# Autodesk Inventor assembly: Hepheaestes38v2 1
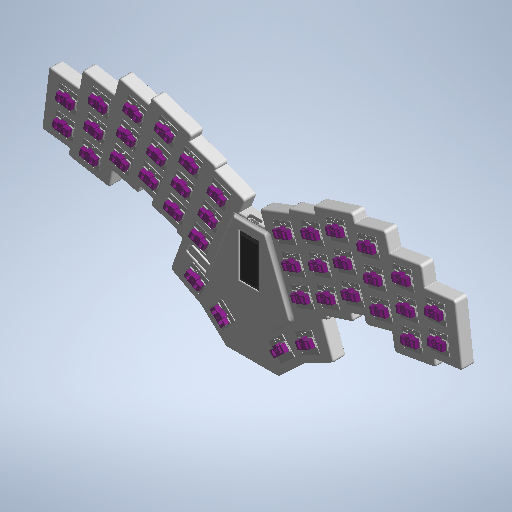
[picture p0: Inventor's stored thumbnail of the model, 512x512]
Saved by Autodesk Inventor 2025 (Build 290162000, 162)
## iProperties
Company: Kicad
Created: 2025-11-22
Part Number: Hepheaestes38v2 1
Description: KiCad electronic assembly
Document SubType Name: Assembly
Designer: User
Authority: Unknown
Mass: 156.593 g
Surface Area: 2055.32 cm^2
Volume: 126.592 cm^3
Density: 1.23699 g/cm^3
Sending System: KiCad to STEP converter
Preprocessor: Open CASCADE STEP processor 7.9
Title: Hepheaestes38v2.step
Author: Pcbnew
## Documents named in this file (18)
- C:\Users\User\Hephaestes38-zmk\PCB, Case\Case V2\Hepheaestes38v2 CAD\Hepheaestes38v2.iam
- C:\Users\User\Hephaestes38-zmk\PCB, Case\Case V2\Hepheaestes38v2 CAD\Hepheaestes38v2_copper.ipt
- C:\Users\User\Hephaestes38-zmk\PCB, Case\Case V2\Hepheaestes38v2 CAD\Hepheaestes38v2_pad.ipt
- C:\Users\User\Hephaestes38-zmk\PCB, Case\Case V2\Hepheaestes38v2 CAD\Hepheaestes38v2_via.ipt
- C:\Users\User\Hephaestes38-zmk\PCB, Case\Case V2\Hepheaestes38v2 CAD\Hepheaestes38v2_silkscreen.ipt
- C:\Users\User\Hephaestes38-zmk\PCB, Case\Case V2\Hepheaestes38v2 CAD\Hepheaestes38v2_PCB.ipt
- C:\Users\User\Hephaestes38-zmk\PCB, Case\Case V2\Hepheaestes38v2 CAD\Nice Nano V2.iam
- C:\Users\User\Hephaestes38-zmk\PCB, Case\Case V2\Hepheaestes38v2 CAD\nice!view\nice!view.ipt
- C:\Users\User\Documents\Inventor\Content Center Files\R2025\en-US\BS EN ISO 7045 Z\EN ISO 7045 - M2 x 5 - 4.8 - Z(1).ipt
- C:\Users\User\Hephaestes38-zmk\PCB, Case\Case V2\Hepheaestes38v2 CAD\PCM12SMTR_PART1.ipt
- C:\Users\User\Hephaestes38-zmk\PCB, Case\Case V2\Hepheaestes38v2 CAD\PTS526 Reset button.ipt
- C:\Users\User\Hephaestes38-zmk\PCB, Case\Case V2\Hepheaestes38v2 CAD\Kailh Choc Hotswap Socket.ipt
- C:\Users\User\Hephaestes38-zmk\PCB, Case\Case V2\Hephaestus38v2 Case Top.ipt
- C:\Users\User\Hephaestes38-zmk\PCB, Case\Case V2\Hephaestus38v2 Case Bottom.ipt
- C:\Users\User\Hephaestes38-zmk\PCB, Case\Case V2\Hephaestus38v2 Switchplate.ipt
- C:\Users\User\Hephaestes38-zmk\PCB, Case\Case V2\Hepheaestes38v2 CAD\S2B-PH-K-S.ipt
- C:\Users\User\Hephaestes38-zmk\PCB, Case\Case V2\Hepheaestes38v2 CAD\Kailh LP Choc Purpz.ipt
- C:\Users\User\Hephaestes38-zmk\PCB, Case\Case V2\Hephaestus38v2 Case Screen Cover.ipt
## Components (100 placed, 17 different names)
1. Nice Nano V2:1 [sub-assembly] — Mate:1, Mate:2, Mate:3
2. nice!view:1 — Mate:4, Mate:5, Mate:6
3. PCM12SMTR_PART1:1 — Mate:60, Mate:61, Mate:62
4. PTS526 Reset button:1 — Mate:63, Flush:1, Flush:2
5. S2B-PH-K-S:1 — Mate:183, Tangent:1
6. Hephaestus38v2 Case Top:1 — Mate:55, Mate:58, Mate:59, Mate:184, Mate:187, Mate:188
7. Hephaestus38v2 Case Bottom:1 — Flush:3, Insert:35, Insert:36, Insert:37, Insert:38, Insert:39, Insert:40, Insert:41, Insert:42, Insert:43, Insert:44
8. Hephaestus38v2 Switchplate:1 — Mate:182, Flush:4, Flush:5
9. Hephaestus38v2 Case Screen Cover:1 — Mate:184, Mate:187, Mate:188
10. 1
11. 2 — Mate:2, Mate:3, Mate:5, Mate:6, Flush:1, Flush:2, Mate:67, Mate:70, Mate:73, Mate:76, Mate:79, Mate:82, Mate:85, Mate:88, Mate:91, Mate:94, Mate:97, Mate:100, Mate:103, Mate:106, Mate:109, Mate:112, Mate:115, Mate:118, Mate:121, Mate:124, Mate:127, Mate:130, Mate:133, Mate:136, Mate:139, Mate:142, Mate:145, Mate:148, Mate:151, Mate:154, Mate:157, Mate:160, Mate:163, Mate:166, Mate:169, Mate:172, Mate:175, Mate:178, Tangent:1
12. 3
13. 4
14. 5 — Mate:1, Mate:4, Mate:7, Mate:8, Mate:9, Mate:10, Mate:11, Mate:12, Insert:1, Insert:2, Insert:3, Insert:4, Insert:5, Insert:6, Insert:7, Insert:8, Insert:9, Insert:10, Insert:11, Insert:12, Insert:13, Insert:14, Mate:13, Mate:14, Mate:15, Mate:16, Mate:17, Mate:18, Mate:19, Mate:20, Mate:21, Mate:22, Mate:23, Mate:24, Mate:25, Mate:26, Insert:15, Insert:16, Insert:17, Insert:18, Insert:19, Mate:28, Insert:20, Insert:22, Insert:23, Insert:21, Mate:29, Mate:30, Mate:31, Mate:32, Mate:33, Mate:34, Mate:35, Mate:36, Mate:37, Mate:38, Mate:39, Mate:40, Mate:41, Mate:42, Insert:24, Insert:25, Insert:26, Insert:27, Insert:28, Insert:29, Insert:30, Insert:31, Insert:32, Insert:33, Insert:34, Mate:43, Mate:44, Mate:45, Mate:46, Mate:47, Mate:48, Mate:49, Mate:50, Mate:51, Mate:52, Mate:53, Mate:55, Mate:58, Mate:59, Mate:60, Mate:61, Mate:62, Mate:63, Mate:65, Mate:66, Mate:68, Mate:69, Mate:71, Mate:72, Mate:74, Mate:75, Mate:77, Mate:78, Mate:80, Mate:81, Mate:83, Mate:84, Mate:86, Mate:87, Mate:89, Mate:90, Mate:92, Mate:93, Mate:95, Mate:96, Mate:98, Mate:99, Mate:101, Mate:102, Mate:104, Mate:105, Mate:107, Mate:108, Mate:110, Mate:111, Mate:113, Mate:114, Mate:116, Mate:117, Mate:119, Mate:120, Mate:122, Mate:123, Mate:125, Mate:126, Mate:128, Mate:129, Mate:131, Mate:132, Mate:134, Mate:135, Mate:137, Mate:138, Mate:140, Mate:141, Mate:143, Mate:144, Mate:146, Mate:147, Mate:149, Mate:150, Mate:152, Mate:153, Mate:155, Mate:156, Mate:158, Mate:159, Mate:161, Mate:162, Mate:164, Mate:165, Mate:167, Mate:168, Mate:170, Mate:171, Mate:173, Mate:174, Mate:176, Mate:177, Insert:45, Mate:183, Flush:4, Flush:5
15. Kailh Choc Hotswap Socket:1 — Mate:65, Mate:66, Mate:67
16. Kailh Choc Hotswap Socket:2 — Mate:68, Mate:69, Mate:70
17. Kailh Choc Hotswap Socket:3 — Mate:74, Mate:75, Mate:76
18. Kailh Choc Hotswap Socket:4 — Mate:77, Mate:78, Mate:79
19. Kailh Choc Hotswap Socket:5 — Mate:71, Mate:72, Mate:73
20. Kailh Choc Hotswap Socket:6 — Mate:83, Mate:84, Mate:85
21. Kailh Choc Hotswap Socket:7 — Mate:89, Mate:90, Mate:91
22. Kailh Choc Hotswap Socket:8 — Mate:80, Mate:81, Mate:82
23. Kailh Choc Hotswap Socket:9 — Mate:86, Mate:87, Mate:88
24. Kailh Choc Hotswap Socket:10 — Mate:92, Mate:93, Mate:94
25. Kailh Choc Hotswap Socket:11 — Mate:95, Mate:96, Mate:97
26. Kailh Choc Hotswap Socket:12 — Mate:98, Mate:99, Mate:100
27. Kailh Choc Hotswap Socket:13 — Mate:101, Mate:102, Mate:103
28. Kailh Choc Hotswap Socket:14 — Mate:104, Mate:105, Mate:106
29. Kailh Choc Hotswap Socket:15 — Mate:107, Mate:108, Mate:109
30. Kailh Choc Hotswap Socket:16 — Mate:110, Mate:111, Mate:112
31. Kailh Choc Hotswap Socket:17 — Mate:113, Mate:114, Mate:115, Flush:3
32. Kailh Choc Hotswap Socket:18 — Mate:116, Mate:117, Mate:118
33. Kailh Choc Hotswap Socket:19 — Mate:119, Mate:120, Mate:121
34. Kailh Choc Hotswap Socket:20 — Mate:122, Mate:123, Mate:124
35. Kailh Choc Hotswap Socket:21 — Mate:125, Mate:126, Mate:127
36. Kailh Choc Hotswap Socket:22 — Mate:128, Mate:129, Mate:130
37. Kailh Choc Hotswap Socket:23 — Mate:131, Mate:132, Mate:133
38. Kailh Choc Hotswap Socket:24 — Mate:134, Mate:135, Mate:136
39. Kailh Choc Hotswap Socket:25 — Mate:137, Mate:138, Mate:139
40. Kailh Choc Hotswap Socket:26 — Mate:140, Mate:141, Mate:142
41. Kailh Choc Hotswap Socket:27 — Mate:143, Mate:144, Mate:145
42. Kailh Choc Hotswap Socket:28 — Mate:146, Mate:147, Mate:148
43. Kailh Choc Hotswap Socket:29 — Mate:155, Mate:156, Mate:157
44. Kailh Choc Hotswap Socket:30 — Mate:152, Mate:153, Mate:154
45. Kailh Choc Hotswap Socket:31 — Mate:149, Mate:150, Mate:151
46. Kailh Choc Hotswap Socket:32 — Mate:161, Mate:162, Mate:163
47. Kailh Choc Hotswap Socket:33 — Mate:164, Mate:165, Mate:166
48. Kailh Choc Hotswap Socket:34 — Mate:167, Mate:168, Mate:169
49. Kailh Choc Hotswap Socket:35 — Mate:170, Mate:171, Mate:172
50. Kailh Choc Hotswap Socket:36 — Mate:158, Mate:159, Mate:160
51. Kailh Choc Hotswap Socket:37 — Mate:173, Mate:174, Mate:175
52. Kailh Choc Hotswap Socket:38 — Mate:176, Mate:177, Mate:178
53. Kailh LP Choc Purpz:1 — Mate:7, Mate:8, Mate:9, Mate:34
54. Kailh LP Choc Purpz:2 — Insert:1, Mate:13
55. Kailh LP Choc Purpz:3 — Mate:10, Mate:11, Mate:12
56. Kailh LP Choc Purpz:4 — Insert:2, Mate:14, Mate:35
57. Kailh LP Choc Purpz:5 — Insert:3, Mate:15, Mate:40
58. Kailh LP Choc Purpz:6 — Insert:4, Mate:16
59. Kailh LP Choc Purpz:7 — Insert:5, Mate:17
60. Kailh LP Choc Purpz:8 — Insert:6, Mate:18
61. Kailh LP Choc Purpz:9 — Insert:7, Mate:19
62. Kailh LP Choc Purpz:10 — Insert:8, Mate:20
63. Kailh LP Choc Purpz:11 — Insert:9, Mate:21
64. Kailh LP Choc Purpz:12 — Insert:10, Mate:22
65. Kailh LP Choc Purpz:13 — Insert:14, Mate:23
66. Kailh LP Choc Purpz:14 — Insert:13, Mate:24
67. Kailh LP Choc Purpz:15 — Insert:12, Mate:25
68. Kailh LP Choc Purpz:16 — Insert:11, Mate:26
69. Kailh LP Choc Purpz:17 — Insert:16, Mate:31
70. Kailh LP Choc Purpz:18 — Insert:23, Mate:30
71. Kailh LP Choc Purpz:19 — Insert:15, Mate:29, Mate:182
72. Kailh LP Choc Purpz:20 — Insert:17, Mate:33
73. Kailh LP Choc Purpz:21 — Insert:18, Mate:36
74. Kailh LP Choc Purpz:22 — Insert:19, Mate:39
75. Kailh LP Choc Purpz:23 — Insert:21, Mate:37
76. Kailh LP Choc Purpz:24 — Insert:22, Mate:32
77. Kailh LP Choc Purpz:25 — Insert:20, Mate:38
78. Kailh LP Choc Purpz:26 — Mate:28, Mate:42
79. Kailh LP Choc Purpz:27 — Mate:41, Insert:45
80. Kailh LP Choc Purpz:28 — Insert:30, Mate:44
81. Kailh LP Choc Purpz:29 — Insert:27, Mate:52
82. Kailh LP Choc Purpz:30 — Insert:24, Mate:49
83. Kailh LP Choc Purpz:31 — Insert:32, Mate:46
84. Kailh LP Choc Purpz:32 — Insert:33, Mate:47
85. Kailh LP Choc Purpz:33 — Insert:34, Mate:48
86. Kailh LP Choc Purpz:34 — Insert:28, Mate:53
87. Kailh LP Choc Purpz:35 — Insert:26, Mate:51
88. Kailh LP Choc Purpz:36 — Insert:25, Mate:50
89. Kailh LP Choc Purpz:37 — Insert:29, Mate:43
90. Kailh LP Choc Purpz:38 — Insert:31, Mate:45
91. BS EN ISO 7045 Z - Metric M2 x 5 - 4.8 - Z:1 — Insert:35
92. BS EN ISO 7045 Z - Metric M2 x 5 - 4.8 - Z:2 — Insert:36
93. BS EN ISO 7045 Z - Metric M2 x 5 - 4.8 - Z:3 — Insert:37
94. BS EN ISO 7045 Z - Metric M2 x 5 - 4.8 - Z:4 — Insert:38
95. BS EN ISO 7045 Z - Metric M2 x 5 - 4.8 - Z:5 — Insert:39
96. BS EN ISO 7045 Z - Metric M2 x 5 - 4.8 - Z:6 — Insert:40
97. BS EN ISO 7045 Z - Metric M2 x 5 - 4.8 - Z:7 — Insert:41
98. BS EN ISO 7045 Z - Metric M2 x 5 - 4.8 - Z:8 — Insert:42
99. BS EN ISO 7045 Z - Metric M2 x 5 - 4.8 - Z:9 — Insert:43
100. BS EN ISO 7045 Z - Metric M2 x 5 - 4.8 - Z:10 — Insert:44
## Relationships (229: Mate 178, Insert 45, Flush 5, Tangent 1)
- Mate:1 (2.54 mm): Nice Nano V2:1 ↔ 5
- Mate:2: Nice Nano V2:1 ↔ 2
- Mate:3: Nice Nano V2:1 ↔ 2
- Mate:4 (5.08 mm): nice!view:1 ↔ 5
- Mate:5: nice!view:1 ↔ 2
- Mate:6: nice!view:1 ↔ 2
- Mate:7: 5 ↔ Kailh LP Choc Purpz:1
- Mate:8: 5 ↔ Kailh LP Choc Purpz:1
- Mate:9: 5 ↔ Kailh LP Choc Purpz:1
- Mate:10: 5 ↔ Kailh LP Choc Purpz:3
- Mate:11: 5 ↔ Kailh LP Choc Purpz:3
- Mate:12: 5 ↔ Kailh LP Choc Purpz:3
- Insert:1: 5 ↔ Kailh LP Choc Purpz:2
- Insert:2: 5 ↔ Kailh LP Choc Purpz:4
- Insert:3: 5 ↔ Kailh LP Choc Purpz:5
- Insert:4: 5 ↔ Kailh LP Choc Purpz:6
- Insert:5: 5 ↔ Kailh LP Choc Purpz:7
- Insert:6: 5 ↔ Kailh LP Choc Purpz:8
- Insert:7: 5 ↔ Kailh LP Choc Purpz:9
- Insert:8: 5 ↔ Kailh LP Choc Purpz:10
- Insert:9: 5 ↔ Kailh LP Choc Purpz:11
- Insert:10: 5 ↔ Kailh LP Choc Purpz:12
- Insert:11: 5 ↔ Kailh LP Choc Purpz:16
- Insert:12: 5 ↔ Kailh LP Choc Purpz:15
- Insert:13: 5 ↔ Kailh LP Choc Purpz:14
- Insert:14: 5 ↔ Kailh LP Choc Purpz:13
- Mate:13: 5 ↔ Kailh LP Choc Purpz:2
- Mate:14: 5 ↔ Kailh LP Choc Purpz:4
- Mate:15: 5 ↔ Kailh LP Choc Purpz:5
- Mate:16: 5 ↔ Kailh LP Choc Purpz:6
- Mate:17: 5 ↔ Kailh LP Choc Purpz:7
- Mate:18: 5 ↔ Kailh LP Choc Purpz:8
- Mate:19: 5 ↔ Kailh LP Choc Purpz:9
- Mate:20: 5 ↔ Kailh LP Choc Purpz:10
- Mate:21: 5 ↔ Kailh LP Choc Purpz:11
- Mate:22: 5 ↔ Kailh LP Choc Purpz:12
- Mate:23: 5 ↔ Kailh LP Choc Purpz:13
- Mate:24: 5 ↔ Kailh LP Choc Purpz:14
- Mate:25: 5 ↔ Kailh LP Choc Purpz:15
- Mate:26: 5 ↔ Kailh LP Choc Purpz:16
- Insert:15: 5 ↔ Kailh LP Choc Purpz:19
- Insert:16: 5 ↔ Kailh LP Choc Purpz:17
- Insert:17: 5 ↔ Kailh LP Choc Purpz:20
- Insert:18: 5 ↔ Kailh LP Choc Purpz:21
- Insert:19: 5 ↔ Kailh LP Choc Purpz:22
- Mate:28: 5 ↔ Kailh LP Choc Purpz:26
- Insert:20: 5 ↔ Kailh LP Choc Purpz:25
- Insert:21: 5 ↔ Kailh LP Choc Purpz:23
- Insert:22: 5 ↔ Kailh LP Choc Purpz:24
- Insert:23: 5 ↔ Kailh LP Choc Purpz:18
- Mate:29: 5 ↔ Kailh LP Choc Purpz:19
- Mate:30: 5 ↔ Kailh LP Choc Purpz:18
- Mate:31: 5 ↔ Kailh LP Choc Purpz:17
- Mate:32: 5 ↔ Kailh LP Choc Purpz:24
- Mate:33: 5 ↔ Kailh LP Choc Purpz:20
- Mate:34: 5 ↔ Kailh LP Choc Purpz:1
- Mate:35: 5 ↔ Kailh LP Choc Purpz:4
- Mate:36: 5 ↔ Kailh LP Choc Purpz:21
- Mate:37: 5 ↔ Kailh LP Choc Purpz:23
- Mate:38: 5 ↔ Kailh LP Choc Purpz:25
- Mate:39: 5 ↔ Kailh LP Choc Purpz:22
- Mate:40: 5 ↔ Kailh LP Choc Purpz:5
- Mate:41: 5 ↔ Kailh LP Choc Purpz:27
- Mate:42: 5 ↔ Kailh LP Choc Purpz:26
- Insert:24: 5 ↔ Kailh LP Choc Purpz:30
- Insert:25: 5 ↔ Kailh LP Choc Purpz:36
- Insert:26: 5 ↔ Kailh LP Choc Purpz:35
- Insert:27: 5 ↔ Kailh LP Choc Purpz:29
- Insert:28: 5 ↔ Kailh LP Choc Purpz:34
- Insert:29: 5 ↔ Kailh LP Choc Purpz:37
- Insert:30: 5 ↔ Kailh LP Choc Purpz:28
- Insert:31: 5 ↔ Kailh LP Choc Purpz:38
- Insert:32: 5 ↔ Kailh LP Choc Purpz:31
- Insert:33: 5 ↔ Kailh LP Choc Purpz:32
- Insert:34: 5 ↔ Kailh LP Choc Purpz:33
- Mate:43: 5 ↔ Kailh LP Choc Purpz:37
- Mate:44: 5 ↔ Kailh LP Choc Purpz:28
- Mate:45: 5 ↔ Kailh LP Choc Purpz:38
- Mate:46: 5 ↔ Kailh LP Choc Purpz:31
- Mate:47: 5 ↔ Kailh LP Choc Purpz:32
- Mate:48: 5 ↔ Kailh LP Choc Purpz:33
- Mate:49: 5 ↔ Kailh LP Choc Purpz:30
- Mate:50: 5 ↔ Kailh LP Choc Purpz:36
- Mate:51: 5 ↔ Kailh LP Choc Purpz:35
- Mate:52: 5 ↔ Kailh LP Choc Purpz:29
- Mate:53: 5 ↔ Kailh LP Choc Purpz:34
- Mate:55: Hephaestus38v2 Case Top:1 ↔ 5
- Mate:58: Hephaestus38v2 Case Top:1 ↔ 5
- Mate:59: Hephaestus38v2 Case Top:1 ↔ 5
- Mate:60: PCM12SMTR_PART1:1 ↔ 5
- Mate:61: PCM12SMTR_PART1:1 ↔ 5
- Mate:62: PCM12SMTR_PART1:1 ↔ 5
- Mate:63: PTS526 Reset button:1 ↔ 5
- Flush:1 (0.5 mm): PTS526 Reset button:1 ↔ 2
- Flush:2 (1 mm): PTS526 Reset button:1 ↔ 2
- Mate:65: 5 ↔ Kailh Choc Hotswap Socket:1
- Mate:66: 5 ↔ Kailh Choc Hotswap Socket:1
- Mate:67: 2 ↔ Kailh Choc Hotswap Socket:1
- Mate:68: 5 ↔ Kailh Choc Hotswap Socket:2
- Mate:69: 5 ↔ Kailh Choc Hotswap Socket:2
- Mate:70: 2 ↔ Kailh Choc Hotswap Socket:2
- Mate:71: 5 ↔ Kailh Choc Hotswap Socket:5
- Mate:72: 5 ↔ Kailh Choc Hotswap Socket:5
- Mate:73: 2 ↔ Kailh Choc Hotswap Socket:5
- Mate:74: 5 ↔ Kailh Choc Hotswap Socket:3
- Mate:75: 5 ↔ Kailh Choc Hotswap Socket:3
- Mate:76: 2 ↔ Kailh Choc Hotswap Socket:3
- Mate:77: 5 ↔ Kailh Choc Hotswap Socket:4
- Mate:78: 5 ↔ Kailh Choc Hotswap Socket:4
- Mate:79: 2 ↔ Kailh Choc Hotswap Socket:4
- Mate:80: 5 ↔ Kailh Choc Hotswap Socket:8
- Mate:81: 5 ↔ Kailh Choc Hotswap Socket:8
- Mate:82: 2 ↔ Kailh Choc Hotswap Socket:8
- Mate:83: 5 ↔ Kailh Choc Hotswap Socket:6
- Mate:84: 5 ↔ Kailh Choc Hotswap Socket:6
- Mate:85: 2 ↔ Kailh Choc Hotswap Socket:6
- Mate:86: 5 ↔ Kailh Choc Hotswap Socket:9
- Mate:87: 5 ↔ Kailh Choc Hotswap Socket:9
- Mate:88: 2 ↔ Kailh Choc Hotswap Socket:9
- Mate:89: 5 ↔ Kailh Choc Hotswap Socket:7
- Mate:90: 5 ↔ Kailh Choc Hotswap Socket:7
- Mate:91: 2 ↔ Kailh Choc Hotswap Socket:7
- Mate:92: 5 ↔ Kailh Choc Hotswap Socket:10
- Mate:93: 5 ↔ Kailh Choc Hotswap Socket:10
- Mate:94: 2 ↔ Kailh Choc Hotswap Socket:10
- Mate:95: 5 ↔ Kailh Choc Hotswap Socket:11
- Mate:96: 5 ↔ Kailh Choc Hotswap Socket:11
- Mate:97: 2 ↔ Kailh Choc Hotswap Socket:11
- Mate:98: 5 ↔ Kailh Choc Hotswap Socket:12
- Mate:99: 5 ↔ Kailh Choc Hotswap Socket:12
- Mate:100: 2 ↔ Kailh Choc Hotswap Socket:12
- Mate:101: 5 ↔ Kailh Choc Hotswap Socket:13
- Mate:102: 5 ↔ Kailh Choc Hotswap Socket:13
- Mate:103: 2 ↔ Kailh Choc Hotswap Socket:13
- Mate:104: 5 ↔ Kailh Choc Hotswap Socket:14
- Mate:105: 5 ↔ Kailh Choc Hotswap Socket:14
- Mate:106: 2 ↔ Kailh Choc Hotswap Socket:14
- Mate:107: 5 ↔ Kailh Choc Hotswap Socket:15
- Mate:108: 5 ↔ Kailh Choc Hotswap Socket:15
- Mate:109: 2 ↔ Kailh Choc Hotswap Socket:15
- Mate:110: 5 ↔ Kailh Choc Hotswap Socket:16
- Mate:111: 5 ↔ Kailh Choc Hotswap Socket:16
- Mate:112: 2 ↔ Kailh Choc Hotswap Socket:16
- Mate:113: 5 ↔ Kailh Choc Hotswap Socket:17
- Mate:114: 5 ↔ Kailh Choc Hotswap Socket:17
- Mate:115: 2 ↔ Kailh Choc Hotswap Socket:17
- Mate:116: 5 ↔ Kailh Choc Hotswap Socket:18
- Mate:117: 5 ↔ Kailh Choc Hotswap Socket:18
- Mate:118: 2 ↔ Kailh Choc Hotswap Socket:18
- Mate:119: 5 ↔ Kailh Choc Hotswap Socket:19
- Mate:120: 5 ↔ Kailh Choc Hotswap Socket:19
- Mate:121: 2 ↔ Kailh Choc Hotswap Socket:19
- Mate:122: 5 ↔ Kailh Choc Hotswap Socket:20
- Mate:123: 5 ↔ Kailh Choc Hotswap Socket:20
- Mate:124: 2 ↔ Kailh Choc Hotswap Socket:20
- Mate:125: 5 ↔ Kailh Choc Hotswap Socket:21
- Mate:126: 5 ↔ Kailh Choc Hotswap Socket:21
- Mate:127: 2 ↔ Kailh Choc Hotswap Socket:21
- Mate:128: 5 ↔ Kailh Choc Hotswap Socket:22
- Mate:129: 5 ↔ Kailh Choc Hotswap Socket:22
- Mate:130: 2 ↔ Kailh Choc Hotswap Socket:22
- Mate:131: 5 ↔ Kailh Choc Hotswap Socket:23
- Mate:132: 5 ↔ Kailh Choc Hotswap Socket:23
- Mate:133: 2 ↔ Kailh Choc Hotswap Socket:23
- Mate:134: 5 ↔ Kailh Choc Hotswap Socket:24
- Mate:135: 5 ↔ Kailh Choc Hotswap Socket:24
- Mate:136: 2 ↔ Kailh Choc Hotswap Socket:24
- Mate:137: 5 ↔ Kailh Choc Hotswap Socket:25
- Mate:138: 5 ↔ Kailh Choc Hotswap Socket:25
- Mate:139: 2 ↔ Kailh Choc Hotswap Socket:25
- Mate:140: 5 ↔ Kailh Choc Hotswap Socket:26
- Mate:141: 5 ↔ Kailh Choc Hotswap Socket:26
- Mate:142: 2 ↔ Kailh Choc Hotswap Socket:26
- Mate:143: 5 ↔ Kailh Choc Hotswap Socket:27
- Mate:144: 5 ↔ Kailh Choc Hotswap Socket:27
- Mate:145: 2 ↔ Kailh Choc Hotswap Socket:27
- Mate:146: 5 ↔ Kailh Choc Hotswap Socket:28
- Mate:147: 5 ↔ Kailh Choc Hotswap Socket:28
- Mate:148: 2 ↔ Kailh Choc Hotswap Socket:28
- Mate:149: 5 ↔ Kailh Choc Hotswap Socket:31
- Mate:150: 5 ↔ Kailh Choc Hotswap Socket:31
- Mate:151: 2 ↔ Kailh Choc Hotswap Socket:31
- Mate:152: 5 ↔ Kailh Choc Hotswap Socket:30
- Mate:153: 5 ↔ Kailh Choc Hotswap Socket:30
- Mate:154: 2 ↔ Kailh Choc Hotswap Socket:30
- Mate:155: 5 ↔ Kailh Choc Hotswap Socket:29
- Mate:156: 5 ↔ Kailh Choc Hotswap Socket:29
- Mate:157: 2 ↔ Kailh Choc Hotswap Socket:29
- Mate:158: 5 ↔ Kailh Choc Hotswap Socket:36
- Mate:159: 5 ↔ Kailh Choc Hotswap Socket:36
- Mate:160: 2 ↔ Kailh Choc Hotswap Socket:36
- Mate:161: 5 ↔ Kailh Choc Hotswap Socket:32
- Mate:162: 5 ↔ Kailh Choc Hotswap Socket:32
- Mate:163: 2 ↔ Kailh Choc Hotswap Socket:32
- Mate:164: 5 ↔ Kailh Choc Hotswap Socket:33
- Mate:165: 5 ↔ Kailh Choc Hotswap Socket:33
- Mate:166: 2 ↔ Kailh Choc Hotswap Socket:33
- Mate:167: 5 ↔ Kailh Choc Hotswap Socket:34
- Mate:168: 5 ↔ Kailh Choc Hotswap Socket:34
- Mate:169: 2 ↔ Kailh Choc Hotswap Socket:34
- Mate:170: 5 ↔ Kailh Choc Hotswap Socket:35
- Mate:171: 5 ↔ Kailh Choc Hotswap Socket:35
- Mate:172: 2 ↔ Kailh Choc Hotswap Socket:35
- Mate:173: 5 ↔ Kailh Choc Hotswap Socket:37
- Mate:174: 5 ↔ Kailh Choc Hotswap Socket:37
- Mate:175: 2 ↔ Kailh Choc Hotswap Socket:37
- Mate:176: 5 ↔ Kailh Choc Hotswap Socket:38
- Mate:177: 5 ↔ Kailh Choc Hotswap Socket:38
- Mate:178: 2 ↔ Kailh Choc Hotswap Socket:38
- Flush:3: Hephaestus38v2 Case Bottom:1 ↔ Kailh Choc Hotswap Socket:17
- Insert:35: Hephaestus38v2 Case Bottom:1 ↔ BS EN ISO 7045 Z - Metric M2 x 5 - 4.8 - Z:1
- Insert:36: Hephaestus38v2 Case Bottom:1 ↔ BS EN ISO 7045 Z - Metric M2 x 5 - 4.8 - Z:2
- Insert:37: Hephaestus38v2 Case Bottom:1 ↔ BS EN ISO 7045 Z - Metric M2 x 5 - 4.8 - Z:3
- Insert:38: Hephaestus38v2 Case Bottom:1 ↔ BS EN ISO 7045 Z - Metric M2 x 5 - 4.8 - Z:4
- Insert:39: Hephaestus38v2 Case Bottom:1 ↔ BS EN ISO 7045 Z - Metric M2 x 5 - 4.8 - Z:5
- Insert:40: Hephaestus38v2 Case Bottom:1 ↔ BS EN ISO 7045 Z - Metric M2 x 5 - 4.8 - Z:6
- Insert:41: Hephaestus38v2 Case Bottom:1 ↔ BS EN ISO 7045 Z - Metric M2 x 5 - 4.8 - Z:7
- Insert:42: Hephaestus38v2 Case Bottom:1 ↔ BS EN ISO 7045 Z - Metric M2 x 5 - 4.8 - Z:8
- Insert:43: Hephaestus38v2 Case Bottom:1 ↔ BS EN ISO 7045 Z - Metric M2 x 5 - 4.8 - Z:9
- Insert:44: Hephaestus38v2 Case Bottom:1 ↔ BS EN ISO 7045 Z - Metric M2 x 5 - 4.8 - Z:10
- Mate:182: Hephaestus38v2 Switchplate:1 ↔ Kailh LP Choc Purpz:19
- Insert:45: 5 ↔ Kailh LP Choc Purpz:27
- Mate:183: S2B-PH-K-S:1 ↔ 5
- Tangent:1: S2B-PH-K-S:1 ↔ 2
- Flush:4: Hephaestus38v2 Switchplate:1 ↔ 5
- Flush:5: Hephaestus38v2 Switchplate:1 ↔ 5
- Mate:184 (0.1 mm): Hephaestus38v2 Case Top:1 ↔ Hephaestus38v2 Case Screen Cover:1
- Mate:187: Hephaestus38v2 Case Top:1 ↔ Hephaestus38v2 Case Screen Cover:1
- Mate:188 (-1 mm): Hephaestus38v2 Case Top:1 ↔ Hephaestus38v2 Case Screen Cover:1
